# Autodesk Inventor assembly: webcam_without_stand
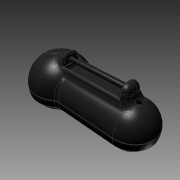
[picture p0: Inventor's stored thumbnail of the model, 180x180]
Saved by Autodesk Inventor 2014 (Build 180170000, 170)
## iProperties
Created: 2011-11-30
Part Number: webcam_without_stand
Document SubType Name: Assembly
Designer: slazh bliskovic
Author: slazh bliskovic
## Documents named in this file (9)
- C:\Users\buben\Documents\GitHub\bacon\inventor files\3rd party components\quickcam pro 9000\webcam_without_stand.iam
- C:\Users\buben\Documents\GitHub\bacon\inventor files\3rd party components\quickcam pro 9000\kamerica.ipt
- C:\Users\buben\Documents\GitHub\bacon\inventor files\3rd party components\quickcam pro 9000\gornji shiny dio.ipt
- C:\Users\buben\Documents\GitHub\bacon\inventor files\3rd party components\quickcam pro 9000\objektiv.ipt
- C:\Users\buben\Documents\GitHub\bacon\inventor files\3rd party components\quickcam pro 9000\unutrasnja plastika.ipt
- C:\Users\buben\Documents\GitHub\bacon\inventor files\3rd party components\quickcam pro 9000\staklence.ipt
- C:\Users\buben\Documents\GitHub\bacon\inventor files\3rd party components\quickcam pro 9000\svjetlasce.ipt
- C:\Users\buben\Documents\GitHub\bacon\inventor files\3rd party components\quickcam pro 9000\staklo.ipt
- C:\Users\buben\Documents\GitHub\bacon\inventor files\3rd party components\quickcam pro 9000\mrezica.ipt
## Components (8 placed, 8 different names)
1. kamerica:1 — Mate:6
2. gornji shiny dio:1 — Angle:1, Mate:6
3. objektiv:1
4. unutrasnja plastika:1
5. staklence:1 — Flush:1
6. svjetlasce:1
7. staklo:1 — Flush:1
8. mrezica:1
## Relationships (4: Mate 2, Flush 1, Angle 1)
- Flush:1 (0.5 mm): staklence:1 ↔ staklo:1
- Mate:4
- Angle:1 (12.5 deg): gornji shiny dio:1
- Mate:6: kamerica:1 ↔ gornji shiny dio:1
